# Autodesk Inventor assembly: Cockpit
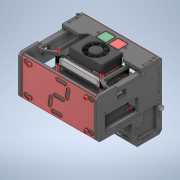
[picture p0: Inventor's stored thumbnail of the model, 180x180]
Saved by Autodesk Inventor 2022.3 (Build 263350000, 350)
## iProperties
Created: 2022-04-25
Part Number: Cockpit
Document SubType Name: Assembly
Designer: Masato Kubotera
Author: Masato Kubotera
## Documents named in this file (25)
- C:\Users\Masato\Desktop\SUSTAINA-OP\UpperBody\Cockpit\Cockpit.iam
- C:\Users\Masato\Desktop\SUSTAINA-OP\UpperBody\Cockpit\Cockpit_circuit_board_frame.ipt
- C:\Users\Masato\Desktop\SUSTAINA-OP\ReadyMade\InsertNut\UD-43040.ipt
- C:\Users\Masato\Desktop\SUSTAINA-OP\UpperBody\Cockpit\Cockpit_front_frame_cloth.ipt
- C:\Users\Masato\Desktop\SUSTAINA-OP\UpperBody\Cockpit\Cockpit_back_frame_cloth.ipt
- C:\Users\Masato\Desktop\SUSTAINA-OP\ElectronicComponents\Board_designed_for_SUSTAINA-OP\SUSTAINA-Core-Board.ipt
- C:\Users\Masato\Desktop\SUSTAINA-OP\UpperBody\Cockpit\SUSTAINA-Core-Board_cover.ipt
- C:\Users\Masato\Desktop\SUSTAINA-OP\ReadyMade\Battery\HP-G830C2800S3.ipt
- C:\Users\Masato\Desktop\SUSTAINA-OP\ReadyMade\Screw\UC-0306.ipt
- C:\Users\Masato\Desktop\SUSTAINA-OP\ReadyMade\Screw\UC-0308.ipt
- C:\Users\Masato\Desktop\SUSTAINA-OP\ElectronicComponents\Board_designed_for_SUSTAINA-OP\Control-Buttons-Module.ipt
- C:\Users\Masato\Desktop\SUSTAINA-OP\ReadyMade\Screw\SPNFL-BRN-M3-10.ipt
- C:\Users\Masato\Desktop\SUSTAINA-OP\UpperBody\Cockpit\Cockpit_carrier_board_frame.iam
- C:\Users\Masato\Desktop\SUSTAINA-OP\UpperBody\Cockpit\Cockpit_top_frame.iam
- C:\Users\Masato\Desktop\SUSTAINA-OP\ElectronicComponents\SingleBoardComputerUnit.iam
- C:\Users\Masato\Desktop\SUSTAINA-OP\UpperBody\Cockpit\Cockpit_from_frame.iam
- C:\Users\Masato\Desktop\SUSTAINA-OP\ReadyMade\Bush\L3040-8110TB.ipt
- C:\Users\Masato\Desktop\SUSTAINA-OP\UpperBody\Cockpit\Cockpit_back_frame.iam
- C:\Users\Masato\Desktop\SUSTAINA-OP\ReadyMade\Screw\UC-2610.ipt
- C:\Users\Masato\Desktop\SUSTAINA-OP\UpperBody\Cockpit\Cockpit_battery_frame.iam
- C:\Users\Masato\Desktop\SUSTAINA-OP\UpperBody\Cockpit\Cockpit_battery_back_door.iam
- C:\Users\Masato\Desktop\SUSTAINA-OP\UpperBody\Cockpit\Cockpit_side_frame.iam
- C:\Users\Masato\Desktop\SUSTAINA-OP\UpperBody\Cockpit\Cockpit_side_frame_MIR.iam
- C:\Users\Masato\Desktop\SUSTAINA-OP\ElectronicComponents\DC-Voltmeter-Red.ipt
- C:\Users\Masato\Desktop\SUSTAINA-OP\UpperBody\Cockpit\Voltmeter_cover.ipt
## Components (72 placed, 24 different names)
1. SUSTAINA-Core-Board:1 — 挿入:63, 挿入:64, 挿入:65, 挿入:66, 挿入:95, 挿入:96, 挿入:166, 挿入:167
2. Control-Buttons-Module:1 — 挿入:105, 挿入:106, 挿入:138, 挿入:139
3. Cockpit_carrier_board_frame:1 [sub-assembly] — 挿入:140, 挿入:141, 挿入:144, 挿入:145, Insert:198, Angle:2
4. Cockpit_carrier_board_frame:2 [sub-assembly] — 挿入:142, 挿入:143, 挿入:146, 挿入:147, Insert:199
5. Cockpit_top_frame:1 [sub-assembly] — 挿入:138, 挿入:139, 挿入:150, 挿入:151, Insert:188, Insert:189
6. SingleBoardComputerUnit:1 [sub-assembly] — 挿入:140, 挿入:141, 挿入:142, 挿入:143
7. UC-0308:13 — 挿入:146
8. UC-0308:14 — 挿入:147
9. Cockpit_from_frame:1 [sub-assembly] — 挿入:156, 挿入:157, 挿入:158, 挿入:159, 挿入:165, Insert:182, Insert:183, Insert:184, Insert:185
10. L3040-8110TB:1 — 挿入:156, 挿入:160, 挿入:164
11. L3040-8110TB:2 — 挿入:157, 挿入:161
12. L3040-8110TB:3 — 挿入:158, 挿入:162
13. L3040-8110TB:4 — 挿入:159, 挿入:163
14. UC-0306:25 — 挿入:160
15. UC-0306:26 — 挿入:161
16. UC-0306:27 — 挿入:162
17. UC-0306:28 — 挿入:163
18. UC-0308:15 — 挿入:166
19. UC-0308:16 — 挿入:167
20. Cockpit_back_frame:1 [sub-assembly] — 挿入:174, 挿入:175, 挿入:176, 挿入:177, 挿入:180, 挿入:181, Insert:190, Insert:191, Insert:192, Insert:193, Insert:218, Insert:219
21. L3040-8110TB:5 — 挿入:174, 挿入:178
22. UC-0306:29
23. L3040-8110TB:6 — 挿入:175, 挿入:179
24. UC-0306:30
25. L3040-8110TB:7 — 挿入:176
26. UC-0306:31
27. L3040-8110TB:8 — 挿入:177
28. UC-0306:32
29. UC-2610:1 — 挿入:180
30. UC-2610:2 — 挿入:181
31. Cockpit_battery_frame:1 [sub-assembly] — Insert:194, Insert:196, Mate:4, Angle:1
32. Cockpit_battery_frame:2 [sub-assembly] — Insert:195, Insert:197, Mate:3
33. Cockpit_battery_back_door:1 [sub-assembly] — Insert:186, Insert:187
34. Cockpit_side_frame:1 [sub-assembly] — Insert:182, Insert:183, Insert:186, Insert:188, Insert:190, Insert:191, Insert:194, Insert:195, Insert:198, Mate:1, Mate:2, Flush:1, Insert:200, Insert:201, Insert:202, Insert:203, Insert:204, Insert:205, Insert:206, Insert:207, Mate:5, Flush:2, Flush:3, Flush:4, Angle:1, Angle:2, Insert:216
35. Cockpit_side_frame_MIR:1 [sub-assembly] — Insert:184, Insert:185, Insert:187, Insert:189, Insert:192, Insert:193, Insert:196, Insert:197, Insert:199, Insert:208, Insert:209, Insert:210, Insert:211, Insert:212, Insert:213, Insert:214, Insert:215, Insert:217
36. UC-0306:34 — Insert:216
37. UC-0306:35 — Insert:217
38. DC-Voltmeter-Red:1 — Insert:218, Insert:219, Insert:220, Insert:221
39. Voltmeter_cover:1 — Insert:220, Insert:221
40. Cockpit_circuit_board_frame:1 — 挿入:55, 挿入:56, 挿入:57, 挿入:58, Mate:1, Mate:2, Flush:1
41. Cockpit_front_frame_cloth:1 — 挿入:164, 挿入:165
42. Cockpit_back_frame_cloth:1 — 挿入:178, 挿入:179
43. SUSTAINA-Core-Board_cover:1 — 挿入:59, 挿入:60, 挿入:61, 挿入:62, 挿入:63, 挿入:64, 挿入:65, 挿入:66
44. UD-43040:5 — 挿入:55, 挿入:59
45. UD-43040:6 — 挿入:56, 挿入:60
46. UD-43040:7 — 挿入:57, 挿入:61
47. UD-43040:8 — 挿入:58, 挿入:62
48. HP-G830C2800S3:1 — Mate:3, Mate:4, Mate:5
49. SPNFL-BRN-M3-10:2 — Insert:215
50. SPNFL-BRN-M3-10:1 — Insert:207
51. UC-0306:1 — Insert:200
52. UC-0306:2 — Insert:202
53. UC-0306:3 — Insert:201
54. UC-0306:5 — Insert:206
55. UC-0306:6 — Insert:205
56. UC-0306:7 — Insert:204
57. UC-0306:8 — Insert:203
58. UC-0306:9 — Insert:208
59. UC-0306:10 — Insert:209
60. UC-0306:11 — Insert:210
61. UC-0306:13 — Insert:212
62. UC-0306:14 — Insert:214
63. UC-0306:15 — Insert:211
64. UC-0306:16 — Insert:213
65. UC-0306:17 — 挿入:105
66. UC-0306:18 — 挿入:106
67. UC-0308:1 — 挿入:144
68. UC-0308:2 — 挿入:145
69. UC-0308:7 — 挿入:95
70. UC-0308:8 — 挿入:96
71. UC-0308:10 — 挿入:150
72. UC-0308:12 — 挿入:151
## Relationships (103: Insert 92, Mate 5, Flush 4, Angle 2)
- 挿入:55 [Insert]: Cockpit_circuit_board_frame:1 ↔ UD-43040:5
- 挿入:56 [Insert]: Cockpit_circuit_board_frame:1 ↔ UD-43040:6
- 挿入:57 [Insert]: Cockpit_circuit_board_frame:1 ↔ UD-43040:7
- 挿入:58 [Insert]: Cockpit_circuit_board_frame:1 ↔ UD-43040:8
- 挿入:59 [Insert]: SUSTAINA-Core-Board_cover:1 ↔ UD-43040:5
- 挿入:60 [Insert]: SUSTAINA-Core-Board_cover:1 ↔ UD-43040:6
- 挿入:61 [Insert]: SUSTAINA-Core-Board_cover:1 ↔ UD-43040:7
- 挿入:62 [Insert]: SUSTAINA-Core-Board_cover:1 ↔ UD-43040:8
- 挿入:63 [Insert]: SUSTAINA-Core-Board:1 ↔ SUSTAINA-Core-Board_cover:1
- 挿入:64 [Insert]: SUSTAINA-Core-Board:1 ↔ SUSTAINA-Core-Board_cover:1
- 挿入:65 [Insert]: SUSTAINA-Core-Board:1 ↔ SUSTAINA-Core-Board_cover:1
- 挿入:66 [Insert]: SUSTAINA-Core-Board:1 ↔ SUSTAINA-Core-Board_cover:1
- 挿入:95 [Insert]: SUSTAINA-Core-Board:1 ↔ UC-0308:7
- 挿入:96 [Insert]: SUSTAINA-Core-Board:1 ↔ UC-0308:8
- 挿入:105 [Insert]: Control-Buttons-Module:1 ↔ UC-0306:17
- 挿入:106 [Insert]: Control-Buttons-Module:1 ↔ UC-0306:18
- 挿入:138 [Insert]: Control-Buttons-Module:1 ↔ Cockpit_top_frame:1
- 挿入:139 [Insert]: Control-Buttons-Module:1 ↔ Cockpit_top_frame:1
- 挿入:140 [Insert]: Cockpit_carrier_board_frame:1 ↔ SingleBoardComputerUnit:1
- 挿入:141 [Insert]: Cockpit_carrier_board_frame:1 ↔ SingleBoardComputerUnit:1
- 挿入:142 [Insert]: Cockpit_carrier_board_frame:2 ↔ SingleBoardComputerUnit:1
- 挿入:143 [Insert]: Cockpit_carrier_board_frame:2 ↔ SingleBoardComputerUnit:1
- 挿入:144 [Insert]: Cockpit_carrier_board_frame:1 ↔ UC-0308:1
- 挿入:145 [Insert]: Cockpit_carrier_board_frame:1 ↔ UC-0308:2
- 挿入:146 [Insert]: Cockpit_carrier_board_frame:2 ↔ UC-0308:13
- 挿入:147 [Insert]: Cockpit_carrier_board_frame:2 ↔ UC-0308:14
- 挿入:150 [Insert]: Cockpit_top_frame:1 ↔ UC-0308:10
- 挿入:151 [Insert]: Cockpit_top_frame:1 ↔ UC-0308:12
- 挿入:156 [Insert]: Cockpit_from_frame:1 ↔ L3040-8110TB:1
- 挿入:157 [Insert]: Cockpit_from_frame:1 ↔ L3040-8110TB:2
- 挿入:158 [Insert]: Cockpit_from_frame:1 ↔ L3040-8110TB:3
- 挿入:159 [Insert]: Cockpit_from_frame:1 ↔ L3040-8110TB:4
- 挿入:160 [Insert]: L3040-8110TB:1 ↔ UC-0306:25
- 挿入:161 [Insert]: L3040-8110TB:2 ↔ UC-0306:26
- 挿入:162 [Insert]: L3040-8110TB:3 ↔ UC-0306:27
- 挿入:163 [Insert]: L3040-8110TB:4 ↔ UC-0306:28
- 挿入:164 [Insert]: L3040-8110TB:1 ↔ Cockpit_front_frame_cloth:1
- 挿入:165 [Insert]: Cockpit_from_frame:1 ↔ Cockpit_front_frame_cloth:1
- 挿入:166 [Insert]: SUSTAINA-Core-Board:1 ↔ UC-0308:15
- 挿入:167 [Insert]: SUSTAINA-Core-Board:1 ↔ UC-0308:16
- [Insert]: L3040-8110TB:5 ↔ UC-0306:29
- [Insert]: L3040-8110TB:6 ↔ UC-0306:30
- [Insert]: L3040-8110TB:7 ↔ UC-0306:31
- [Insert]: L3040-8110TB:8 ↔ UC-0306:32
- 挿入:174 [Insert]: Cockpit_back_frame:1 ↔ L3040-8110TB:5
- 挿入:175 [Insert]: Cockpit_back_frame:1 ↔ L3040-8110TB:6
- 挿入:176 [Insert]: Cockpit_back_frame:1 ↔ L3040-8110TB:7
- 挿入:177 [Insert]: Cockpit_back_frame:1 ↔ L3040-8110TB:8
- 挿入:178 [Insert]: L3040-8110TB:5 ↔ Cockpit_back_frame_cloth:1
- 挿入:179 [Insert]: L3040-8110TB:6 ↔ Cockpit_back_frame_cloth:1
- 挿入:180 [Insert]: Cockpit_back_frame:1 ↔ UC-2610:1
- 挿入:181 [Insert]: Cockpit_back_frame:1 ↔ UC-2610:2
- Insert:182: Cockpit_from_frame:1 ↔ Cockpit_side_frame:1
- Insert:183: Cockpit_from_frame:1 ↔ Cockpit_side_frame:1
- Insert:184: Cockpit_from_frame:1 ↔ Cockpit_side_frame_MIR:1
- Insert:185: Cockpit_from_frame:1 ↔ Cockpit_side_frame_MIR:1
- Insert:186: Cockpit_battery_back_door:1 ↔ Cockpit_side_frame:1
- Insert:187: Cockpit_battery_back_door:1 ↔ Cockpit_side_frame_MIR:1
- Insert:188: Cockpit_top_frame:1 ↔ Cockpit_side_frame:1
- Insert:189: Cockpit_top_frame:1 ↔ Cockpit_side_frame_MIR:1
- Insert:190: Cockpit_back_frame:1 ↔ Cockpit_side_frame:1
- Insert:191: Cockpit_back_frame:1 ↔ Cockpit_side_frame:1
- Insert:192: Cockpit_back_frame:1 ↔ Cockpit_side_frame_MIR:1
- Insert:193: Cockpit_back_frame:1 ↔ Cockpit_side_frame_MIR:1
- Insert:194: Cockpit_battery_frame:1 ↔ Cockpit_side_frame:1
- Insert:195: Cockpit_battery_frame:2 ↔ Cockpit_side_frame:1
- Insert:196: Cockpit_battery_frame:1 ↔ Cockpit_side_frame_MIR:1
- Insert:197: Cockpit_battery_frame:2 ↔ Cockpit_side_frame_MIR:1
- Insert:198: Cockpit_carrier_board_frame:1 ↔ Cockpit_side_frame:1
- Insert:199: Cockpit_carrier_board_frame:2 ↔ Cockpit_side_frame_MIR:1
- Mate:1 (0.05 mm): Cockpit_side_frame:1 ↔ Cockpit_circuit_board_frame:1
- Mate:2 (0.05 mm): Cockpit_side_frame:1 ↔ Cockpit_circuit_board_frame:1
- Flush:1: Cockpit_side_frame:1 ↔ Cockpit_circuit_board_frame:1
- Insert:200: Cockpit_side_frame:1 ↔ UC-0306:1
- Insert:201: Cockpit_side_frame:1 ↔ UC-0306:3
- Insert:202: Cockpit_side_frame:1 ↔ UC-0306:2
- Insert:203: Cockpit_side_frame:1 ↔ UC-0306:8
- Insert:204: Cockpit_side_frame:1 ↔ UC-0306:7
- Insert:205: Cockpit_side_frame:1 ↔ UC-0306:6
- Insert:206: Cockpit_side_frame:1 ↔ UC-0306:5
- Insert:207: Cockpit_side_frame:1 ↔ SPNFL-BRN-M3-10:1
- Insert:208: Cockpit_side_frame_MIR:1 ↔ UC-0306:9
- Insert:209: Cockpit_side_frame_MIR:1 ↔ UC-0306:10
- Insert:210: Cockpit_side_frame_MIR:1 ↔ UC-0306:11
- Insert:211: Cockpit_side_frame_MIR:1 ↔ UC-0306:15
- Insert:212: Cockpit_side_frame_MIR:1 ↔ UC-0306:13
- Insert:213: Cockpit_side_frame_MIR:1 ↔ UC-0306:16
- Insert:214: Cockpit_side_frame_MIR:1 ↔ UC-0306:14
- Insert:215: Cockpit_side_frame_MIR:1 ↔ SPNFL-BRN-M3-10:2
- Mate:3: Cockpit_battery_frame:2 ↔ HP-G830C2800S3:1
- Mate:4: Cockpit_battery_frame:1 ↔ HP-G830C2800S3:1
- Mate:5: Cockpit_side_frame:1 ↔ HP-G830C2800S3:1
- Flush:2: Cockpit_side_frame:1
- Flush:3 (67.5 mm): Cockpit_side_frame:1
- Flush:4: Cockpit_side_frame:1
- Angle:1 (0 deg): Cockpit_battery_frame:1 ↔ Cockpit_side_frame:1
- Angle:2 (0 deg): Cockpit_carrier_board_frame:1 ↔ Cockpit_side_frame:1
- Insert:216: Cockpit_side_frame:1 ↔ UC-0306:34
- Insert:217: Cockpit_side_frame_MIR:1 ↔ UC-0306:35
- Insert:218: Cockpit_back_frame:1 ↔ DC-Voltmeter-Red:1
- Insert:219: Cockpit_back_frame:1 ↔ DC-Voltmeter-Red:1
- Insert:220: DC-Voltmeter-Red:1 ↔ Voltmeter_cover:1
- Insert:221: DC-Voltmeter-Red:1 ↔ Voltmeter_cover:1
## Named parameters: d215_d205 = 0 mm, d216_d205 = 0 mm, d217_d205 = 0 mm, d218_d205 = 0 mm
